# Autodesk Inventor assembly: Assembly2
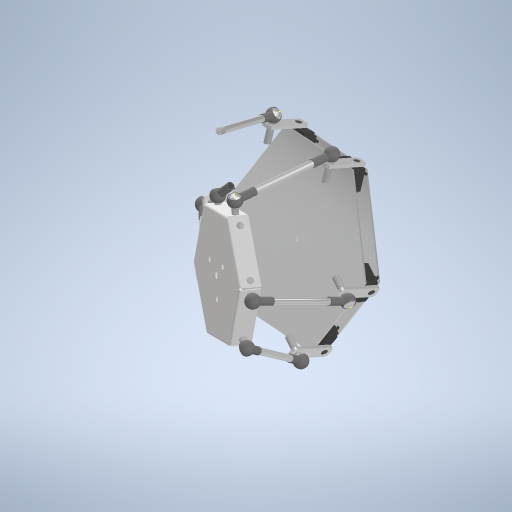
[picture p0: Inventor's stored thumbnail of the model, 512x512]
Saved by Autodesk Inventor 2023 (Build 270158000, 158)
## iProperties
Created: 2022-06-30
Part Number: Assembly2
Document SubType Name: Assembly
Designer: earls
Author: earls
## Documents named in this file (6)
- F:\Documents\Mechatronic Engineering 5.1\Project\CAD\Assembly2.iam
- F:\Documents\Mechatronic Engineering 5.1\Project\CAD\Moving platform.ipt
- F:\Documents\Mechatronic Engineering 5.1\Project\CAD\Spherical joint\Part2.ipt
- F:\Documents\Mechatronic Engineering 5.1\Project\CAD\Spherical joint\Part1.ipt
- F:\Documents\Mechatronic Engineering 5.1\Project\CAD\Stewart Assembly.iam
- F:\Documents\Mechatronic Engineering 5.1\Project\CAD\Rod qty-6.ipt
## Components (32 placed, 5 different names)
1. Moving platform:1 — Insert:2, Insert:4, Insert:6, Insert:13, Insert:14, Insert:15
2. Part2:1 — Insert:15, Ball:21
3. Part2:2 — Insert:2, Ball:17
4. Part2:3 — Insert:13, Ball:18
5. Part2:4 — Insert:4, Ball:20
6. Part2:5 — Insert:14, Ball:19
7. Part2:6 — Insert:6, Ball:22
8. Part1:1 — Ball:20, Mate:11, Mate:12
9. Part1:3 — Ball:19, Mate:15
10. Part1:4 — Ball:22, Mate:7, Mate:8
11. Part1:5 — Ball:21, Mate:3, Mate:4
12. Stewart Assembly:1 [sub-assembly] — Insert:7, Insert:8, Insert:9, Insert:10, Insert:11, Insert:12
13. Part2:7 — Insert:9, Ball:7
14. Part2:8 — Insert:7, Ball:12
15. Part2:9 — Insert:11, Ball:13
16. Part2:10 — Insert:8, Ball:11
17. Part2:11 — Insert:10, Ball:8
18. Part2:13 — Insert:12, Ball:9
19. Part1:7 — Ball:12, Mate:16, Mate:17
20. Part1:8 — Ball:9, Mate:1, Mate:2
21. Part1:9 — Ball:13, Mate:5, Mate:6
22. Part1:10 — Ball:11, Mate:19, Mate:20
23. Part1:11 — Ball:8, Mate:13, Mate:14
24. Part1:12 — Ball:7, Mate:9, Mate:10
25. Part1:13 — Ball:17, Mate:18, Mate:21
26. Part1:14 — Ball:18
27. Rod qty-6:1 — Mate:9, Mate:10, Mate:11, Mate:12
28. Rod qty-6:2 — Mate:13, Mate:14, Mate:15
29. Rod qty-6:3 — Mate:1, Mate:2, Mate:3, Mate:4
30. Rod qty-6:4 — Mate:16, Mate:17, Mate:18, Mate:21
31. Rod qty-6:5 — Mate:19, Mate:20
32. Rod qty-6:7 — Mate:5, Mate:6, Mate:7, Mate:8
## Relationships (45: Mate 21, Insert 12, BallJoint 12)
- Insert:2 (-10 mm): Moving platform:1 ↔ Part2:2
- Insert:4 (-10 mm): Moving platform:1 ↔ Part2:4
- Insert:6 (-10 mm): Moving platform:1 ↔ Part2:6
- Insert:7 (-3 mm): Stewart Assembly:1 ↔ Part2:8
- Insert:8 (-3 mm): Stewart Assembly:1 ↔ Part2:10
- Insert:9 (-3 mm): Stewart Assembly:1 ↔ Part2:7
- Insert:10 (-3 mm): Stewart Assembly:1 ↔ Part2:11
- Insert:11 (-3 mm): Stewart Assembly:1 ↔ Part2:9
- Insert:12 (-3 mm): Stewart Assembly:1 ↔ Part2:13
- Ball:7: Part2:7 ↔ Part1:12
- Ball:8: Part2:11 ↔ Part1:11
- Ball:9: Part2:13 ↔ Part1:8
- Ball:11: Part2:10 ↔ Part1:10
- Ball:12: Part2:8 ↔ Part1:7
- Ball:13: Part2:9 ↔ Part1:9
- Insert:13 (-3 mm): Moving platform:1 ↔ Part2:3
- Ball:17: Part2:2 ↔ Part1:13
- Ball:18: Part2:3 ↔ Part1:14
- Insert:14 (-3 mm): Moving platform:1 ↔ Part2:5
- Ball:19: Part2:5 ↔ Part1:3
- Ball:20: Part2:4 ↔ Part1:1
- Insert:15 (-3 mm): Moving platform:1 ↔ Part2:1
- Ball:21: Part2:1 ↔ Part1:5
- Mate:1: Part1:8 ↔ Rod qty-6:3
- Mate:2: Part1:8 ↔ Rod qty-6:3
- Mate:3: Part1:5 ↔ Rod qty-6:3
- Mate:4: Part1:5 ↔ Rod qty-6:3
- Ball:22: Part2:6 ↔ Part1:4
- Mate:5: Part1:9 ↔ Rod qty-6:7
- Mate:6: Part1:9 ↔ Rod qty-6:7
- Mate:7: Part1:4 ↔ Rod qty-6:7
- Mate:8: Part1:4 ↔ Rod qty-6:7
- Mate:9: Part1:12 ↔ Rod qty-6:1
- Mate:10: Part1:12 ↔ Rod qty-6:1
- Mate:11: Part1:1 ↔ Rod qty-6:1
- Mate:12: Part1:1 ↔ Rod qty-6:1
- Mate:13: Part1:11 ↔ Rod qty-6:2
- Mate:14: Part1:11 ↔ Rod qty-6:2
- Mate:15: Part1:3 ↔ Rod qty-6:2
- Mate:16: Part1:7 ↔ Rod qty-6:4
- Mate:17: Part1:7 ↔ Rod qty-6:4
- Mate:18: Part1:13 ↔ Rod qty-6:4
- Mate:19: Part1:10 ↔ Rod qty-6:5
- Mate:20: Part1:10 ↔ Rod qty-6:5
- Mate:21: Part1:13 ↔ Rod qty-6:4
